# Autodesk Inventor assembly: Claw Assembly
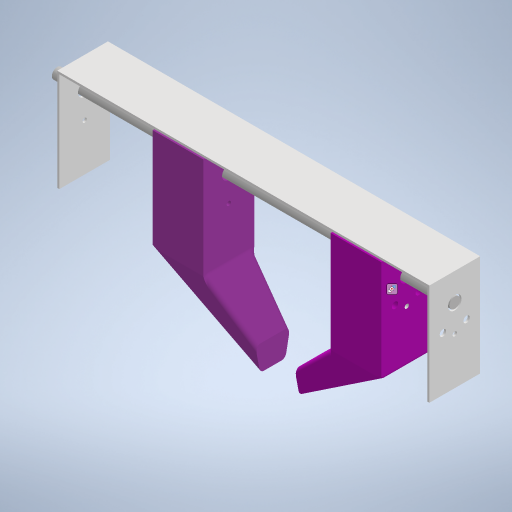
[picture p0: Inventor's stored thumbnail of the model, 512x512]
Saved by Autodesk Inventor 2024 (Build 280153000, 153)
## iProperties
Created: 2025-01-21
Part Number: Claw Assembly
Document SubType Name: Assembly
Designer: Sven
Author: Sven
## Documents named in this file (5)
- C:\Users\Sven\Documents\Inventor\BRC Robotic CLaw\Claw Assembly.iam
- C:\Users\Sven\Documents\Inventor\BRC Robotic CLaw\Bracket.ipt
- C:\Users\Sven\Documents\Inventor\BRC Robotic CLaw\Moving Gripper.ipt
- C:\Users\Sven\Documents\Inventor\BRC Robotic CLaw\Stationary Gripper.ipt
- C:\Users\Sven\Documents\Inventor\BRC Robotic CLaw\Lead Screw.ipt
## Components (4 placed, 4 different names)
1. Bracket:1 — Mate:3, Flush:1, Mate:4, Mate:5
2. Moving Gripper:1 — Mate:5, Mate:6
3. Stationary Gripper:1 — Mate:4, Mate:7
4. Lead Screw:1 — Mate:3, Flush:1, Mate:6, Mate:7
## Relationships (6: Mate 5, Flush 1)
- Mate:3: Bracket:1 ↔ Lead Screw:1
- Flush:1: Bracket:1 ↔ Lead Screw:1
- Mate:4: Bracket:1 ↔ Stationary Gripper:1
- Mate:5: Bracket:1 ↔ Moving Gripper:1
- Mate:6: Moving Gripper:1 ↔ Lead Screw:1
- Mate:7: Stationary Gripper:1 ↔ Lead Screw:1
